# Autodesk Inventor assembly: Biblow Assssssssemblee
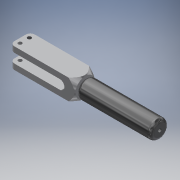
[picture p0: Inventor's stored thumbnail of the model, 180x180]
Saved by Autodesk Inventor 2017 (Build 210142000, 142)
## iProperties
Created: 2017-04-21
Part Number: Biblow Assssssssemblee
Document SubType Name: Assembly
Designer: 193515
Author: 193515
## Documents named in this file (5)
- C:\Users\193515.FCBOE.000\Desktop\Biblow Assssssssemblee.iam
- C:\Users\193515.FCBOE.000\Documents\Part1.ipt
- C:\Users\193515.FCBOE.000\Desktop\handle bar.ipt
- C:\Users\193515.FCBOE.000\Desktop\middle handle piece (hard).ipt
- C:\Users\193515.FCBOE.000\Desktop\Part2.ipt
## Components (4 placed, 4 different names)
1. Part1:1 — Rigid:1
2. middle handle piece (hard):1 — Rigid:1, Rotational:1
3. Part2:1 — Rotational:1, Rotational:2
4. handle bar:1 — Rotational:2
## Relationships (3: RevoluteJoint 2, WeldJoint 1)
- Rigid:1 [WeldJoint]: Part1:1 ↔ middle handle piece (hard):1
- Rotational:1 [RevoluteJoint]: middle handle piece (hard):1 ↔ Part2:1
- Rotational:2 [RevoluteJoint]: Part2:1 ↔ handle bar:1
